# Autodesk Inventor assembly: lazer_boi
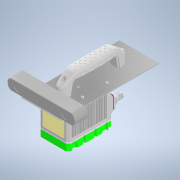
[picture p0: Inventor's stored thumbnail of the model, 180x180]
Saved by Autodesk Inventor 2021 (Build 250183000, 183)
## iProperties
Created: 2020-08-20
Part Number: lazer_boi
Document SubType Name: Assembly
Designer: Haden
Author: Haden
## Documents named in this file (9)
- C:\Users\Haden\Documents\GitHub\1k-nm-boi\lazer_boi.iam
- C:\Users\Haden\Documents\GitHub\1k-nm-boi\ZED\ZED.ipt
- C:\Users\Haden\Documents\GitHub\1k-nm-boi\Handle.ipt
- C:\Users\Haden\Documents\GitHub\1k-nm-boi\Fasteners\1 inch quarter 20 bolt.ipt
- C:\Users\Haden\Documents\GitHub\1k-nm-boi\Fasteners\Quarter 20 locknut.ipt
- C:\Users\Haden\Documents\GitHub\1k-nm-boi\Fasteners\M3 standoff.ipt
- C:\Users\Haden\Documents\GitHub\1k-nm-boi\Fasteners\M3x6 bolt.ipt
- C:\Users\Haden\Documents\GitHub\1k-nm-boi\Aluminum Plate.ipt
- C:\Users\Haden\Documents\GitHub\1k-nm-boi\LiDAR.iam
## Components (20 placed, 8 different names)
1. LiDAR:1 [sub-assembly] — Insert:1, Insert:2, Insert:3, Insert:4, Insert:5, Insert:6, Angle:2
2. M3 standoff:1 — Insert:1, Flush:1, Angle:1, Insert:8
3. M3 standoff:2 — Insert:2, Flush:3, Angle:1, Angle:2, Insert:7
4. M3 standoff:3 — Insert:4, Flush:3, Flush:4
5. M3 standoff:4 — Insert:3, Flush:1, Flush:2
6. M3 standoff:5 — Insert:5, Flush:4
7. M3 standoff:6 — Insert:6, Flush:2
8. M3x6 bolt:1 — Insert:9
9. M3x6 bolt:2 — Insert:11
10. M3x6 bolt:3 — Insert:14
11. M3x6 bolt:4 — Insert:10
12. M3x6 bolt:5 — Insert:12
13. M3x6 bolt:6 — Insert:13
14. Aluminum Plate:1 — Insert:7, Insert:8, Insert:9, Insert:10, Insert:11, Insert:12, Insert:13, Insert:14, Mate:1, Angle:3, Mate:2, Insert:15, Insert:16, Insert:19, Insert:20
15. ZED:1 — Mate:1, Angle:3, Mate:2
16. Handle:1 — Insert:17, Insert:18, Insert:19, Insert:20
17. 1 inch quarter 20 bolt:1 — Insert:17
18. 1 inch quarter 20 bolt:2 — Insert:18
19. Quarter 20 locknut:1 — Insert:15
20. Quarter 20 locknut:2 — Insert:16
## Relationships (29: Insert 20, Flush 4, Angle 3, Mate 2)
- Insert:1: LiDAR:1 ↔ M3 standoff:1
- Insert:2: LiDAR:1 ↔ M3 standoff:2
- Insert:3: LiDAR:1 ↔ M3 standoff:4
- Insert:4: LiDAR:1 ↔ M3 standoff:3
- Insert:5: LiDAR:1 ↔ M3 standoff:5
- Insert:6: LiDAR:1 ↔ M3 standoff:6
- Flush:1: M3 standoff:1 ↔ M3 standoff:4
- Flush:2: M3 standoff:4 ↔ M3 standoff:6
- Flush:3: M3 standoff:2 ↔ M3 standoff:3
- Flush:4: M3 standoff:3 ↔ M3 standoff:5
- Angle:1 (0 deg): M3 standoff:1 ↔ M3 standoff:2
- Angle:2 (0 deg): LiDAR:1 ↔ M3 standoff:2
- Insert:7: M3 standoff:2 ↔ Aluminum Plate:1
- Insert:8: M3 standoff:1 ↔ Aluminum Plate:1
- Insert:9: M3x6 bolt:1 ↔ Aluminum Plate:1
- Insert:10: M3x6 bolt:4 ↔ Aluminum Plate:1
- Insert:11: M3x6 bolt:2 ↔ Aluminum Plate:1
- Insert:12: M3x6 bolt:5 ↔ Aluminum Plate:1
- Insert:13: M3x6 bolt:6 ↔ Aluminum Plate:1
- Insert:14: M3x6 bolt:3 ↔ Aluminum Plate:1
- Mate:1: Aluminum Plate:1 ↔ ZED:1
- Angle:3 (0 deg): Aluminum Plate:1 ↔ ZED:1
- Mate:2: Aluminum Plate:1 ↔ ZED:1
- Insert:15: Aluminum Plate:1 ↔ Quarter 20 locknut:1
- Insert:16: Aluminum Plate:1 ↔ Quarter 20 locknut:2
- Insert:17: Handle:1 ↔ 1 inch quarter 20 bolt:1
- Insert:18: Handle:1 ↔ 1 inch quarter 20 bolt:2
- Insert:19: Aluminum Plate:1 ↔ Handle:1
- Insert:20: Aluminum Plate:1 ↔ Handle:1
